# Autodesk Inventor assembly: omniwheel_MIR
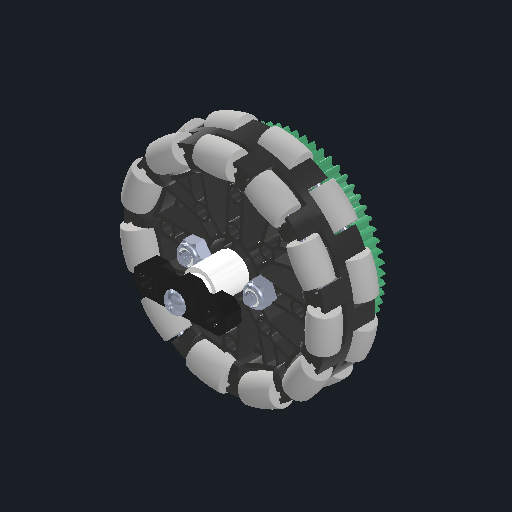
[picture p0: Inventor's stored thumbnail of the model, 512x512]
Saved by Autodesk Inventor 2024 (Build 280153000, 153)
## iProperties
Created: 2023-08-09
Part Number: omniwheel_MIR
Document SubType Name: Assembly
Designer: macbook
Author: macbook
## Documents named in this file (13)
- \\Mac\Home\Desktop\code\1599V-VRC\Cad\Assembly\v3\omniwheel_MIR.iam
- \\Mac\Home\Desktop\code\1599V-VRC\Cad\Motion\Wheels\Omni Wheel\3.25 Omni AS, cir_MIR2.iam
- \\Mac\Home\Desktop\code\1599V-VRC\Cad\Structure\Hardware\Nut Nylock_MIR7.ipt
- \\Mac\Home\Desktop\code\1599V-VRC\Cad\Motion\Shaft LS\Bearing Flat_MIR7.ipt
- \\Mac\Home\Desktop\code\1599V-VRC\Cad\Structure\Hardware\Screw Steel - Star\SScrew Star Smooth 2.500.ipt
- \\Mac\Home\Desktop\code\1599V-VRC\Cad\Structure\Hardware\Screw Steel - Star.ipt
- \\Mac\Home\Desktop\code\1599V-VRC\Cad\Motion\Spacers\Spacer Nylon .500 OD\NSpacer White .500 OD x .500.ipt
- \\Mac\Home\Desktop\code\1599V-VRC\Cad\Motion\Spacers\Spacer Nylon .500 OD.ipt
- \\Mac\Home\Desktop\code\1599V-VRC\Cad\Motion\Gears\LS 60T Gear_MIR5.ipt
- \\Mac\Home\Desktop\code\1599V-VRC\Cad\Motion\Spacers\Spacer Nylon .500 OD\NSpacer White .500 OD x .375.ipt
- \\Mac\Home\Desktop\code\1599V-VRC\Cad\Structure\Hardware\Screw Steel - Star\SScrew Star Threaded 1.250.ipt
- \\Mac\Home\Desktop\code\1599V-VRC\Cad\Motion\Spacers\Washer Teflon\TWasher .375 OD x .06250.ipt
- \\Mac\Home\Desktop\code\1599V-VRC\Cad\Motion\Spacers\Washer Teflon.ipt
## Components (15 placed, 9 different names)
1. 3.25 Omni AS, cir_MIR2:1 [sub-assembly] — Insert:117, Insert:118, Insert:132, Insert:130, Insert:131
2. Nut Nylock_MIR7:1 — Insert:117
3. Nut Nylock_MIR7:2 — Insert:118
4. Bearing Flat_MIR7:1 — Insert:120, Insert:119, Insert:122
5. Bearing Flat_MIR7:2 — Insert:120, Insert:119, Insert:121, Insert:134
6. SScrew Star Smooth 2.500:1 — Insert:121
7. Nut Nylock_MIR7:3 — Insert:122
8. NSpacer White .500 OD x .500:1 — Insert:132, Insert:133
9. LS 60T Gear_MIR5:1 — Insert:129, Insert:126, Insert:127, Insert:128, Insert:135
10. NSpacer White .500 OD x .375:2 — Insert:130, Insert:129
11. NSpacer White .500 OD x .375:3 — Insert:131, Insert:126
12. SScrew Star Threaded 1.250:2 — Insert:127
13. SScrew Star Threaded 1.250:3 — Insert:128
14. TWasher .375 OD x .06250:1 — Insert:134, Insert:133
15. TWasher .375 OD x .06250:2 — Insert:135
## Relationships (16: Insert 16)
- Insert:117: 3.25 Omni AS, cir_MIR2:1 ↔ Nut Nylock_MIR7:1
- Insert:118: 3.25 Omni AS, cir_MIR2:1 ↔ Nut Nylock_MIR7:2
- Insert:120 (44.45 mm): Bearing Flat_MIR7:1 ↔ Bearing Flat_MIR7:2
- Insert:119 (44.45 mm): Bearing Flat_MIR7:1 ↔ Bearing Flat_MIR7:2
- Insert:121 (1.5875 mm): Bearing Flat_MIR7:2 ↔ SScrew Star Smooth 2.500:1
- Insert:122: Bearing Flat_MIR7:1 ↔ Nut Nylock_MIR7:3
- Insert:132: 3.25 Omni AS, cir_MIR2:1 ↔ NSpacer White .500 OD x .500:1
- Insert:130: 3.25 Omni AS, cir_MIR2:1 ↔ NSpacer White .500 OD x .375:2
- Insert:129: LS 60T Gear_MIR5:1 ↔ NSpacer White .500 OD x .375:2
- Insert:131: 3.25 Omni AS, cir_MIR2:1 ↔ NSpacer White .500 OD x .375:3
- Insert:126: LS 60T Gear_MIR5:1 ↔ NSpacer White .500 OD x .375:3
- Insert:127: LS 60T Gear_MIR5:1 ↔ SScrew Star Threaded 1.250:2
- Insert:128: LS 60T Gear_MIR5:1 ↔ SScrew Star Threaded 1.250:3
- Insert:134: Bearing Flat_MIR7:2 ↔ TWasher .375 OD x .06250:1
- Insert:133: NSpacer White .500 OD x .500:1 ↔ TWasher .375 OD x .06250:1
- Insert:135: LS 60T Gear_MIR5:1 ↔ TWasher .375 OD x .06250:2
